# Autodesk Inventor assembly: Marker Changer - Spiny Parts
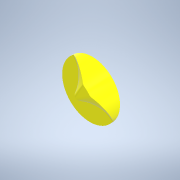
[picture p0: Inventor's stored thumbnail of the model, 180x180]
Saved by Autodesk Inventor 2022.2 (Build 262287000, 287)
## iProperties
Created: 2022-02-09
Part Number: Marker Changer - Spiny Parts
Document SubType Name: Assembly
Designer: smiku
Author: smiku
## Documents named in this file (3)
- C:\Users\smiku\3D Objects\GrabCAD\AACC Mechatonics Capstone\Marker Changer\Subassemblies\Marker Changer - Spiny Parts.iam
- C:\Users\smiku\3D Objects\GrabCAD\AACC Mechatonics Capstone\Marker Changer\Single Cam Plate.ipt
- C:\Users\smiku\3D Objects\GrabCAD\AACC Mechatonics Capstone\Interface\Servo\Servo Hub.ipt
## Components (2 placed, 2 different names)
1. Servo Hub:1 — Rigid:1
2. Single Cam Plate:1 — Rigid:1
## Relationships (1: WeldJoint 1)
- Rigid:1 [WeldJoint]: Servo Hub:1 ↔ Single Cam Plate:1
